# Autodesk Inventor assembly: !Second Stage
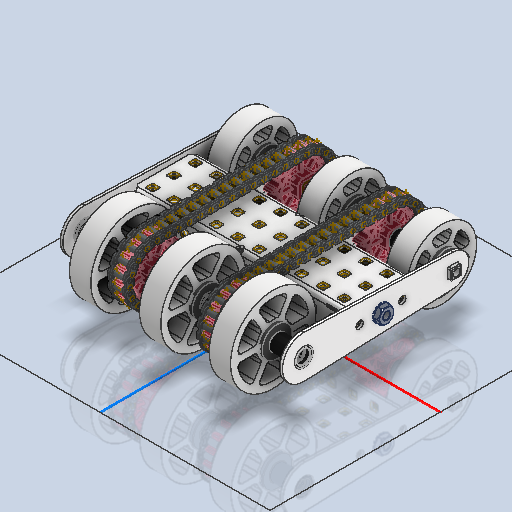
[picture p0: Inventor's stored thumbnail of the model, 512x512]
Saved by Autodesk Inventor 2026 (Build 300175000, 175)
## iProperties
Created: 2025-04-12
Part Number: !Second Stage
Document SubType Name: Assembly
Designer: avere
Author: avere
## Documents named in this file (25)
- C:\Users\avere\OneDrive\Documents\VEX-CAD\V5-CAD\Floating Stage\Second Stage\!Second Stage.iam
- C:\Users\avere\OneDrive\Documents\VEX-CAD\V5-CAD\Floating Stage\Second Stage\Custom Parts\Gusset.ipt
- C:\Users\avere\OneDrive\Documents\VEX-CAD\VEX-CAD-Inventor\Structure\Angle\Aluminum 1x1\Alu Angle 1x1x3.ipt
- C:\Users\avere\OneDrive\Documents\VEX-CAD\VEX-CAD-Inventor\Motion\Shaft HS\HS Bushing 0.1250.ipt
- C:\Users\avere\OneDrive\Documents\VEX-CAD\VEX-CAD-Inventor\Motion\Insert Circle.ipt
- C:\Users\avere\OneDrive\Documents\VEX-CAD\VEX-CAD-Inventor\Structure\C Channel\Aluminum 1x3x1\Alu C 1x3x1x10.ipt
- C:\Users\avere\OneDrive\Documents\VEX-CAD\VEX-CAD-Inventor\Motion\Wheels\Flex Wheels\1.625 Flex Wheel\1.625 30A .500.ipt
- C:\Users\avere\OneDrive\Documents\VEX-CAD\VEX-CAD-Inventor\Motion\Wheels\Flex Wheels\1.625 Flex Wheel.ipt
- C:\Users\avere\OneDrive\Documents\VEX-CAD\VEX-CAD-Inventor\Motion\Wheels\Flex Wheels\VersaHex Adapters .250.ipt
- C:\Users\avere\OneDrive\Documents\VEX-CAD\VEX-CAD-Inventor\Motion\Insert Square.ipt
- C:\Users\avere\OneDrive\Documents\VEX-CAD\VEX-CAD-Inventor\Motion\Spacers\Spacer Nylon .375 OD.ipt
- C:\Users\avere\OneDrive\Documents\VEX-CAD\VEX-CAD-Inventor\Motion\Sprockets\6P Sprocket\6P 16T Sprocket, No Insert.iam
- C:\Users\avere\OneDrive\Documents\VEX-CAD\VEX-CAD-Inventor\Motion\Sprockets\6P Sprocket.iam
- C:\Users\avere\OneDrive\Documents\VEX-CAD\VEX-CAD-Inventor\Motion\Wheels\Flex Wheels\2.000 Flex Wheel\2.000 30A .500.ipt
- C:\Users\avere\OneDrive\Documents\VEX-CAD\VEX-CAD-Inventor\Motion\Wheels\Flex Wheels\2.000 Flex Wheel.ipt
- C:\Users\avere\OneDrive\Documents\VEX-CAD\VEX-CAD-Inventor\Motion\Shaft HS\HS Spacer\HSpacer .5000.ipt
- C:\Users\avere\OneDrive\Documents\VEX-CAD\VEX-CAD-Inventor\Motion\Shaft HS\HS Spacer.ipt
- C:\Users\avere\OneDrive\Documents\VEX-CAD\VEX-CAD-Inventor\Motion\Shaft HS\HS Spacer\HSpacer .1250.ipt
- C:\Users\avere\OneDrive\Documents\VEX-CAD\VEX-CAD-Inventor\Motion\Shaft HS\HS Spacer\HSpacer .2500.ipt
- C:\Users\avere\OneDrive\Documents\VEX-CAD\VEX-CAD-Inventor\Motion\Shaft HS\HS Spacer\HSpacer .0625.ipt
- C:\Users\avere\OneDrive\Documents\VEX-CAD\VEX-CAD-Inventor\Motion\Spacers\Spacer Nylon .375 OD\NSpacer .375 OD x .375.ipt
- C:\Users\avere\OneDrive\Documents\VEX-CAD\VEX-CAD-Inventor\Motion\Spacers\Washer Steel\SWasher .375 OD x .031250.ipt
- C:\Users\avere\OneDrive\Documents\VEX-CAD\VEX-CAD-Inventor\Motion\Spacers\Washer Steel.ipt
- C:\Users\avere\OneDrive\Documents\VEX-CAD\VEX-CAD-Inventor\Structure\Hardware\Nut Keps.ipt
- C:\Users\avere\OneDrive\Documents\VEX-CAD\V5-CAD\Floating Stage\Second Stage\Chain Generator 6P (16x16x3.500204347).ipt
## Components (53 placed, 18 different names)
1. Gusset:1 — Insert:1, Mate:1, Insert:2, Mate:2, Mate:3, Mate:4, Insert:53
2. Alu Angle 1x1x3:1 — Insert:1, Mate:1, Insert:3, Mate:8
3. HS Bushing 0.1250:1 — Insert:2, Insert:32
4. Insert Circle:1 — Mate:2, Mate:3, Mate:4, Insert:10
5. Alu C 1x3x1x10:1 — Mate:5, Mate:6, Flush:1, Mate:7, Insert:3, Mate:8, Insert:11, Mate:13
6. Gusset:2 — Mate:10, Mate:11, Mate:12, Insert:5, Insert:12, Mate:14, Insert:52
7. Alu Angle 1x1x3:2 — Insert:11, Mate:13, Insert:12, Mate:14
8. HS Bushing 0.1250:2 — Insert:5, Insert:30
9. Insert Circle:2 — Mate:10, Mate:11, Mate:12, Insert:23
10. 1.625 30A .500:1 — Insert:6, Insert:7, Mate:18
11. VersaHex Adapters .250:1 — Insert:7, Insert:9
12. VersaHex Adapters .250:2 — Insert:6, Insert:8
13. Insert Square:1 — Insert:9
14. Insert Square:2 — Insert:8, Insert:10
15. 6P 16T Sprocket, No Insert:2 [sub-assembly] — Flush:3, Insert:39, Insert:54
16. 1.625 30A .500:2 — Insert:16, Insert:17
17. VersaHex Adapters .250:3 — Insert:16, Insert:18
18. VersaHex Adapters .250:4 — Insert:17, Insert:19
19. Insert Square:3 — Insert:18, Mate:20
20. Insert Square:4 — Insert:19, Insert:23
21. VersaHex Adapters .250:5 — Insert:33
22. VersaHex Adapters .250:6 — Mate:16, Insert:34
23. 2.000 30A .500:1
24. HSpacer .5000:1 — Insert:32, Insert:33
25. VersaHex Adapters .250:7 — Insert:46
26. VersaHex Adapters .250:8 — Insert:31
27. 2.000 30A .500:2
28. HSpacer .5000:2 — Insert:30, Insert:31
29. VersaHex Adapters .250:9
30. VersaHex Adapters .250:10
31. 2.000 30A .500:3 — Flush:2
32. 6P 16T Sprocket, No Insert:4 [sub-assembly] — Mate:16, Flush:3, Insert:34, Insert:37
33. HSpacer .2500:4 — Insert:35
34. HSpacer .0625:5 — Insert:36, Insert:37
35. HSpacer .1250:6 — Insert:35, Insert:36
36. NSpacer .375 OD x .375:5 — Insert:38, Insert:39
37. SWasher .375 OD x .031250:1 — Insert:38
38. 6P 16T Sprocket, No Insert:5 [sub-assembly] — Flush:4, Insert:45, Insert:55
39. 6P 16T Sprocket, No Insert:6 [sub-assembly] — Flush:4, Insert:46, Insert:47
40. HSpacer .2500:7 — Insert:42, Insert:47, Mate:19
41. HSpacer .0625:8 — Insert:41
42. HSpacer .1250:9 — Insert:41, Insert:42
43. NSpacer .375 OD x .375:6 — Insert:44, Insert:45, Mate:20
44. SWasher .375 OD x .031250:2 — Insert:44
45. 1.625 30A .500:3 — Mate:17
46. VersaHex Adapters .250:11
47. VersaHex Adapters .250:12 — Mate:18
48. Insert Square:5
49. Insert Square:6
50. Nut Keps:1 — Insert:53
51. Nut Keps:2 — Insert:52
52. Chain Generator 6P (16x16x3.500204347):1 — Insert:54
53. Chain Generator 6P (16x16x3.500204347):2 — Insert:55, Mate:19
## Relationships (69: Insert 46, Mate 19, Flush 4)
- Insert:1: Gusset:1 ↔ Alu Angle 1x1x3:1
- Mate:1: Gusset:1 ↔ Alu Angle 1x1x3:1
- Insert:2: Gusset:1 ↔ HS Bushing 0.1250:1
- Mate:2: Gusset:1 ↔ Insert Circle:1
- Mate:3: Gusset:1 ↔ Insert Circle:1
- Mate:4: Gusset:1 ↔ Insert Circle:1
- Mate:5: Alu C 1x3x1x10:1
- Mate:6: Alu C 1x3x1x10:1
- Flush:1: Alu C 1x3x1x10:1
- Mate:7: Alu C 1x3x1x10:1
- Insert:3: Alu Angle 1x1x3:1 ↔ Alu C 1x3x1x10:1
- Mate:8: Alu Angle 1x1x3:1 ↔ Alu C 1x3x1x10:1
- Mate:10: Gusset:2 ↔ Insert Circle:2
- Mate:11: Gusset:2 ↔ Insert Circle:2
- Mate:12: Gusset:2 ↔ Insert Circle:2
- Insert:5: Gusset:2 ↔ HS Bushing 0.1250:2
- Insert:6: 1.625 30A .500:1 ↔ VersaHex Adapters .250:2
- Insert:7: 1.625 30A .500:1 ↔ VersaHex Adapters .250:1
- Insert:8: VersaHex Adapters .250:2 ↔ Insert Square:2
- Insert:9: VersaHex Adapters .250:1 ↔ Insert Square:1
- Insert:10: Insert Circle:1 ↔ Insert Square:2
- Insert:11: Alu C 1x3x1x10:1 ↔ Alu Angle 1x1x3:2
- Mate:13: Alu C 1x3x1x10:1 ↔ Alu Angle 1x1x3:2
- Insert:12: Gusset:2 ↔ Alu Angle 1x1x3:2
- Mate:14: Gusset:2 ↔ Alu Angle 1x1x3:2
- Insert:16: 1.625 30A .500:2 ↔ VersaHex Adapters .250:3
- Insert:17: 1.625 30A .500:2 ↔ VersaHex Adapters .250:4
- Insert:18: VersaHex Adapters .250:3 ↔ Insert Square:3
- Insert:19: VersaHex Adapters .250:4 ↔ Insert Square:4
- Insert:23: Insert Circle:2 ↔ Insert Square:4
- [Insert]: VersaHex Adapters .250:5 ↔ 2.000 30A .500:1
- [Insert]: VersaHex Adapters .250:6 ↔ 2.000 30A .500:1
- [Insert]: VersaHex Adapters .250:7 ↔ 2.000 30A .500:2
- [Insert]: VersaHex Adapters .250:8 ↔ 2.000 30A .500:2
- [Insert]: VersaHex Adapters .250:9 ↔ 2.000 30A .500:3
- [Insert]: VersaHex Adapters .250:10 ↔ 2.000 30A .500:3
- [Mate]: HSpacer .5000:2 ↔ VersaHex Adapters .250:9
- Insert:30: HS Bushing 0.1250:2 ↔ HSpacer .5000:2
- Insert:31: VersaHex Adapters .250:8 ↔ HSpacer .5000:2
- Insert:32: HS Bushing 0.1250:1 ↔ HSpacer .5000:1
- Insert:33: VersaHex Adapters .250:5 ↔ HSpacer .5000:1
- Flush:2 (-6.35 mm): 2.000 30A .500:3
- Mate:16: VersaHex Adapters .250:6 ↔ 6P 16T Sprocket, No Insert:4
- Flush:3: 6P 16T Sprocket, No Insert:2 ↔ 6P 16T Sprocket, No Insert:4
- Insert:34: VersaHex Adapters .250:6 ↔ 6P 16T Sprocket, No Insert:4
- Insert:35: HSpacer .2500:4 ↔ HSpacer .1250:6
- Insert:36: HSpacer .0625:5 ↔ HSpacer .1250:6
- Insert:37: 6P 16T Sprocket, No Insert:4 ↔ HSpacer .0625:5
- Insert:38: NSpacer .375 OD x .375:5 ↔ SWasher .375 OD x .031250:1
- Insert:39: 6P 16T Sprocket, No Insert:2 ↔ NSpacer .375 OD x .375:5
- Flush:4: 6P 16T Sprocket, No Insert:5 ↔ 6P 16T Sprocket, No Insert:6
- Insert:41: HSpacer .0625:8 ↔ HSpacer .1250:9
- Insert:42: HSpacer .2500:7 ↔ HSpacer .1250:9
- Insert:44: NSpacer .375 OD x .375:6 ↔ SWasher .375 OD x .031250:2
- Insert:45: 6P 16T Sprocket, No Insert:5 ↔ NSpacer .375 OD x .375:6
- Insert:46: VersaHex Adapters .250:7 ↔ 6P 16T Sprocket, No Insert:6
- Insert:47: 6P 16T Sprocket, No Insert:6 ↔ HSpacer .2500:7
- [Insert]: 1.625 30A .500:3 ↔ VersaHex Adapters .250:12
- [Insert]: 1.625 30A .500:3 ↔ VersaHex Adapters .250:11
- [Insert]: VersaHex Adapters .250:12 ↔ Insert Square:6
- [Insert]: VersaHex Adapters .250:11 ↔ Insert Square:5
- Mate:17 (-6.35 mm): 1.625 30A .500:3
- Mate:18: 1.625 30A .500:1 ↔ VersaHex Adapters .250:12
- Insert:52: Gusset:2 ↔ Nut Keps:2
- Insert:53: Gusset:1 ↔ Nut Keps:1
- Insert:54 (-6.35 mm): 6P 16T Sprocket, No Insert:2 ↔ Chain Generator 6P (16x16x3.500204347):1
- Insert:55 (-6.35 mm): 6P 16T Sprocket, No Insert:5 ↔ Chain Generator 6P (16x16x3.500204347):2
- Mate:19: HSpacer .2500:7 ↔ Chain Generator 6P (16x16x3.500204347):2
- Mate:20: Insert Square:3 ↔ NSpacer .375 OD x .375:6
## Named parameters: d81_d71 = 0 mm, d82_d72 = 0 mm, d87_d85 = 0 mm, d88_d86 = 0 mm, d70_d19 = 0 mm, d71_d20 = 0 mm, d72_d21 = 0 mm, d73_d22 = 0 mm
